# Autodesk Inventor assembly: Lower Goal
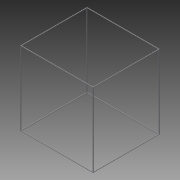
[picture p0: Inventor's stored thumbnail of the model, 180x180]
Saved by Autodesk Inventor 2014 (Build 180170000, 170)
## iProperties
Created: 2014-01-29
Part Number: Lower Goal
Document SubType Name: Assembly
Designer: NilesStanton
Author: NilesStanton
## Documents named in this file (5)
- C:\GitHub\team3566-2014\CAD\Court\Lower Goal.iam
- C:\GitHub\team3566-2014\CAD\Court\Lower Goal Longer.ipt
- C:\GitHub\team3566-2014\CAD\Court\Part4.ipt
- H:\Part1.ipt
- C:\GitHub\team3566-2014\CAD\Court\Part3.ipt
## Components (13 placed, 4 different names)
1. Lower Goal Longer:1 — Flush:1, Flush:2, Flush:3, Flush:4, Flush:5, Flush:6
2. Lower Goal Longer:2 — Flush:7, Flush:8, Flush:9
3. Part4:1 — Flush:4, Flush:5, Flush:6, Mate:3, Mate:4
4. Part4:2 — Flush:1, Flush:2, Flush:3, Flush:7, Flush:8, Flush:9
5. Lower Goal Longer:3 — Mate:6, Mate:9
6. Lower Goal Longer:4 — Mate:2, Mate:11
7. Part4:3 — Mate:1, Mate:5, Mate:7
8. Part4:4 — Mate:8, Mate:10
9. Part1:1
10. Part3:1 — Mate:5, Mate:6, Mate:7
11. Part3:2 — Mate:1, Mate:2, Mate:3, Mate:4
12. Part3:3 — Mate:10, Mate:11
13. Part3:4 — Mate:8, Mate:9
## Relationships (29: Flush 18, Mate 11)
- Flush:1: Lower Goal Longer:1 ↔ Part4:2
- Flush:2: Lower Goal Longer:1 ↔ Part4:2
- Flush:3: Lower Goal Longer:1 ↔ Part4:2
- Flush:4: Lower Goal Longer:1 ↔ Part4:1
- Flush:5: Lower Goal Longer:1 ↔ Part4:1
- Flush:6: Lower Goal Longer:1 ↔ Part4:1
- Flush:7: Lower Goal Longer:2 ↔ Part4:2
- Flush:8: Lower Goal Longer:2 ↔ Part4:2
- Flush:9: Lower Goal Longer:2 ↔ Part4:2
- [Flush]: Lower Goal Longer:3 ↔ Part4:4
- [Flush]: Lower Goal Longer:3 ↔ Part4:4
- [Flush]: Lower Goal Longer:3 ↔ Part4:4
- [Flush]: Lower Goal Longer:3 ↔ Part4:3
- [Flush]: Lower Goal Longer:3 ↔ Part4:3
- [Flush]: Lower Goal Longer:3 ↔ Part4:3
- [Flush]: Lower Goal Longer:4 ↔ Part4:4
- [Flush]: Lower Goal Longer:4 ↔ Part4:4
- [Flush]: Lower Goal Longer:4 ↔ Part4:4
- Mate:1: Part4:3 ↔ Part3:2
- Mate:2: Lower Goal Longer:4 ↔ Part3:2
- Mate:3: Part4:1 ↔ Part3:2
- Mate:4: Part4:1 ↔ Part3:2
- Mate:5: Part4:3 ↔ Part3:1
- Mate:6: Lower Goal Longer:3 ↔ Part3:1
- Mate:7: Part4:3 ↔ Part3:1
- Mate:8: Part4:4 ↔ Part3:4
- Mate:9: Lower Goal Longer:3 ↔ Part3:4
- Mate:10: Part4:4 ↔ Part3:3
- Mate:11: Lower Goal Longer:4 ↔ Part3:3
## Named parameters: d30_d26 = 0 mm, d31_d27 = 0 mm, d32_d28 = 0 mm, d33_d29 = 0 mm, d34_d21 = 0 mm, d35_d22 = 0 mm, d36_d23 = 0 mm, d37_d24 = 0 mm, d38_d25 = 0 mm
